# Autodesk Inventor assembly: HbSensorU02
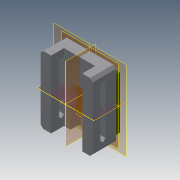
[picture p0: Inventor's stored thumbnail of the model, 180x180]
Saved by Autodesk Inventor 2015 SP1 (Build 190203100, 203)
## iProperties
Created: 2016-01-28
Part Number: HbSensorU02
Document SubType Name: Assembly
Designer: Yamaura
Author: Yamaura
## Documents named in this file (3)
- C:\Users\Yamaura\Documents\GitHub\HACKberry\HACKberry-hardware\3D\Inventor\Parts\HbSensorU02.iam
- C:\Users\Yamaura\Documents\GitHub\HACKberry\HACKberry-hardware\3D\Inventor\Parts\HbSensorBoard02.ipt
- C:\Users\Yamaura\Documents\GitHub\HACKberry\HACKberry-hardware\3D\Inventor\Parts\HbSensorHolder02.ipt
## Components (2 placed, 2 different names)
1. HbSensorBoard02:1 — メイト:1, メイト:2, メイト:3
2. HbSensorHolder02:1 — メイト:1, メイト:2, メイト:3
## Relationships (3: Mate 3)
- メイト:1 [Mate]: HbSensorBoard02:1 ↔ HbSensorHolder02:1
- メイト:2 [Mate]: HbSensorBoard02:1 ↔ HbSensorHolder02:1
- メイト:3 [Mate]: HbSensorBoard02:1 ↔ HbSensorHolder02:1
